# Autodesk Inventor assembly: Geneva Drive and Frame Assembly
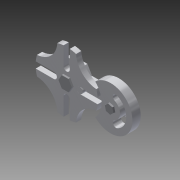
[picture p0: Inventor's stored thumbnail of the model, 180x180]
Saved by Autodesk Inventor 2018 (Build 220112000, 112)
## iProperties
Created: 2018-01-19
Part Number: Geneva Drive and Frame Assembly
Document SubType Name: Assembly
Designer: Rus
Author: Rus
## Documents named in this file (6)
- E:\Libraries\3D Objects\Geneva drive\Mechanical\Attempt 2v3 Simple\Geneva Drive and Frame Assembly.iam
- E:\Libraries\3D Objects\Geneva drive\Mechanical\Attempt 2v3 Simple\Geneva Drive.ipt
- E:\Libraries\3D Objects\Geneva drive\Mechanical\Attempt 2v3 Simple\Geneva Driven.ipt
- E:\Libraries\3D Objects\Geneva drive\Mechanical\Attempt 2v3 Simple\Frame.ipt
- E:\Libraries\3D Objects\Geneva drive\Mechanical\Attempt 2v3 Simple\Driver Shaft Cap.ipt
- E:\Libraries\3D Objects\Geneva drive\Mechanical\Attempt 2v2\Driven Pin.ipt
## Components (5 placed, 5 different names)
1. Geneva Drive:1 — Rotational:1, Mate:1, Mate:2
2. Geneva Driven:1 — Insert:1, Angle:2
3. Frame:1 — Insert:1, Insert:2, Rotational:1, Insert:3, Angle:1
4. Driver Shaft Cap:1 — Insert:3
5. Driven Pin:1 — Insert:2
## Relationships (8: Insert 3, Mate 2, Angle 2, RevoluteJoint 1)
- Insert:1: Geneva Driven:1 ↔ Frame:1
- Insert:2: Frame:1 ↔ Driven Pin:1
- Rotational:1 [RevoluteJoint]: Geneva Drive:1 ↔ Frame:1
- Insert:3: Frame:1 ↔ Driver Shaft Cap:1
- Mate:1: Geneva Drive:1
- Mate:2: Geneva Drive:1
- Angle:1 (0 deg): Frame:1
- Angle:2 (0 deg): Geneva Driven:1
